# Autodesk Inventor assembly: SEPARACION LATA-BOTELLA Y PAPEL
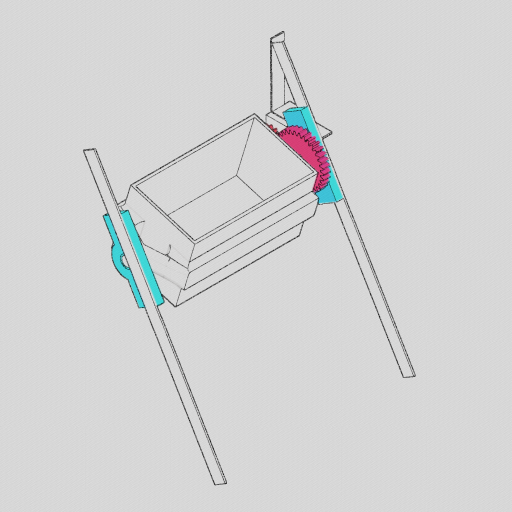
[picture p0: Inventor's stored thumbnail of the model, 512x512]
Saved by Autodesk Inventor 2024 (Build 280153000, 153)
## iProperties
Created: 2024-06-16
Part Number: SEPARACION LATA-BOTELLA Y PAPEL
Document SubType Name: Assembly
Designer: Jhuliams
Author: Jhuliams
## Documents named in this file (9)
- C:\Users\Jhuliams\Documents\GitHub\RECICLADOR_MODELO_3D\MECANISMO DE COMPACTADO\SEPARACION LATA-BOTELLA Y PAPEL.iam
- C:\Users\Jhuliams\Documents\GitHub\RECICLADOR_MODELO_3D\MECANISMO DE COMPACTADO\CAJA PARA DETECCION DE OBJETO.ipt
- C:\Users\Jhuliams\Documents\GitHub\RECICLADOR_MODELO_3D\MECANISMO DE COMPACTADO\ENGRANAJE CONDUCTOR DE CAJA.ipt
- C:\Users\Jhuliams\Documents\GitHub\RECICLADOR_MODELO_3D\MECANISMO DE COMPACTADO\ENGRANE MOTRIZ DE CAJA.ipt
- C:\Users\Jhuliams\Documents\GitHub\RECICLADOR_MODELO_3D\MECANISMO DE COMPACTADO\SOPORTE DE CAJA SEPARADORA.ipt
- C:\Users\Jhuliams\Documents\GitHub\RECICLADOR_MODELO_3D\MECANISMO DE COMPACTADO\NEMA 17 PARA TAPA PRINCIPAL.ipt
- C:\Users\Jhuliams\Documents\GitHub\RECICLADOR_MODELO_3D\MECANISMO DE COMPACTADO\PLETINA PARA CAJA.ipt
- C:\Users\Jhuliams\Documents\GitHub\RECICLADOR_MODELO_3D\MECANISMO DE COMPACTADO\SOPORTE DE NEMA.ipt
- C:\Users\Jhuliams\Documents\GitHub\RECICLADOR_MODELO_3D\MECANISMO DE COMPACTADO\PLETINA NEMA CAJA.ipt
## Components (10 placed, 8 different names)
1. NEMA 17 PARA TAPA PRINCIPAL:1 — Mate:1, Mate:2, Mate:11, Mate:12, Flush:7
2. ENGRANE MOTRIZ DE CAJA:1 — Mate:1, Mate:2, Flush:1, Mate:3, Rotation:1
3. ENGRANAJE CONDUCTOR DE CAJA:1 — Flush:1, Mate:3, Mate:4, Rotation:1, Mate:5, Flush:2, Mate:6
4. CAJA PARA DETECCION DE OBJETO:1 — Mate:5, Flush:2, Mate:6, Flush:3, Mate:7, Mate:8, Flush:4
5. SOPORTE DE CAJA SEPARADORA:1 — Flush:3, Mate:7, Mate:9, Flush:5
6. SOPORTE DE CAJA SEPARADORA:2 — Mate:8, Flush:4, Mate:10, Flush:6
7. PLETINA PARA CAJA:1 — Mate:9, Flush:5
8. PLETINA PARA CAJA:2 — Mate:10, Flush:6, Mate:14
9. SOPORTE DE NEMA:1 — Mate:11, Mate:12, Flush:7, Mate:13, Flush:8
10. PLETINA NEMA CAJA:1 — Mate:13, Mate:14, Flush:8
## Relationships (23: Mate 14, Flush 8, RelateRotation 1)
- Mate:1: NEMA 17 PARA TAPA PRINCIPAL:1 ↔ ENGRANE MOTRIZ DE CAJA:1
- Mate:2: NEMA 17 PARA TAPA PRINCIPAL:1 ↔ ENGRANE MOTRIZ DE CAJA:1
- Flush:1: ENGRANE MOTRIZ DE CAJA:1 ↔ ENGRANAJE CONDUCTOR DE CAJA:1
- Mate:3 (70.5 mm): ENGRANE MOTRIZ DE CAJA:1 ↔ ENGRANAJE CONDUCTOR DE CAJA:1
- Mate:4: ENGRANAJE CONDUCTOR DE CAJA:1
- Rotation:1 [RelateRotation] (0.4242 ul): ENGRANE MOTRIZ DE CAJA:1 ↔ ENGRANAJE CONDUCTOR DE CAJA:1
- Mate:5: ENGRANAJE CONDUCTOR DE CAJA:1 ↔ CAJA PARA DETECCION DE OBJETO:1
- Flush:2: ENGRANAJE CONDUCTOR DE CAJA:1 ↔ CAJA PARA DETECCION DE OBJETO:1
- Mate:6: ENGRANAJE CONDUCTOR DE CAJA:1 ↔ CAJA PARA DETECCION DE OBJETO:1
- Flush:3: CAJA PARA DETECCION DE OBJETO:1 ↔ SOPORTE DE CAJA SEPARADORA:1
- Mate:7: CAJA PARA DETECCION DE OBJETO:1 ↔ SOPORTE DE CAJA SEPARADORA:1
- Mate:8: CAJA PARA DETECCION DE OBJETO:1 ↔ SOPORTE DE CAJA SEPARADORA:2
- Flush:4: CAJA PARA DETECCION DE OBJETO:1 ↔ SOPORTE DE CAJA SEPARADORA:2
- Mate:9: SOPORTE DE CAJA SEPARADORA:1 ↔ PLETINA PARA CAJA:1
- Flush:5: SOPORTE DE CAJA SEPARADORA:1 ↔ PLETINA PARA CAJA:1
- Mate:10: SOPORTE DE CAJA SEPARADORA:2 ↔ PLETINA PARA CAJA:2
- Flush:6: SOPORTE DE CAJA SEPARADORA:2 ↔ PLETINA PARA CAJA:2
- Mate:11: NEMA 17 PARA TAPA PRINCIPAL:1 ↔ SOPORTE DE NEMA:1
- Mate:12: NEMA 17 PARA TAPA PRINCIPAL:1 ↔ SOPORTE DE NEMA:1
- Flush:7: NEMA 17 PARA TAPA PRINCIPAL:1 ↔ SOPORTE DE NEMA:1
- Mate:13: SOPORTE DE NEMA:1 ↔ PLETINA NEMA CAJA:1
- Mate:14: PLETINA PARA CAJA:2 ↔ PLETINA NEMA CAJA:1
- Flush:8: SOPORTE DE NEMA:1 ↔ PLETINA NEMA CAJA:1
